# Autodesk Inventor assembly: s-assy-base_light
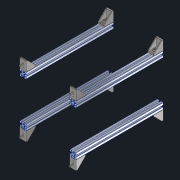
[picture p0: Inventor's stored thumbnail of the model, 180x180]
Saved by Autodesk Inventor 2022 (Build 260153000, 153)
## iProperties
Created: 2021-10-19
Part Number: s-assy-base_light
Document SubType Name: Assembly
Designer: Yuta Kage
Mass: 997.591 g
Surface Area: 2388.51 cm^2
Volume: 260.269 cm^3
Density: 3.83292 g/cm^3
Author: Yuta Kage
## Documents named in this file (4)
- C:\Users\yuta0\Documents\GitHub\catchrobo_hardware\assy-scara\s-assy-base_light.iam
- C:\Users\yuta0\Documents\GitHub\catchrobo_hardware\assy-scara\NFS5-2020_1.ipt
- C:\Users\yuta0\Documents\GitHub\catchrobo_hardware\assy-scara\s-assy-blacket2.iam
- C:\Users\yuta0\Documents\GitHub\catchrobo_hardware\assy-scara\CB5-15.ipt
## Components (16 placed, 3 different names)
1. CB5-15:1
2. CB5-15:2
3. CB5-15:3
4. CB5-15:4
5. s-assy-blacket2:2 [sub-assembly] — メイト:19, フラッシュ:25, フラッシュ:26
6. NFS5-2020_1:5 — メイト:18, フラッシュ:23, フラッシュ:24, メイト:19, フラッシュ:25, フラッシュ:26
7. s-assy-blacket2:1 [sub-assembly] — メイト:18, フラッシュ:23, フラッシュ:24
8. NFS5-2020_1:3 — フラッシュ:28, メイト:21, フラッシュ:29, フラッシュ:30, メイト:25, フラッシュ:31
9. s-assy-blacket2:3 [sub-assembly] — フラッシュ:28, メイト:25, フラッシュ:31
10. s-assy-blacket2:7 [sub-assembly] — メイト:21, フラッシュ:29, フラッシュ:30
11. s-assy-blacket2:8 [sub-assembly]
12. NFS5-2020_1:6
13. s-assy-blacket2:9 [sub-assembly]
14. NFS5-2020_1:7
15. s-assy-blacket2:10 [sub-assembly]
16. s-assy-blacket2:11 [sub-assembly]
## Component patterns: (4 elements, first: CB5-15:1), (2 elements, first: s-assy-blacket2:2 + NFS5-2020_1:5 + s-assy-blacket2:1 + NFS5-2020_1:3 + s-assy-blacket2:3 + s-assy-blacket2:7)
## Relationships (12: Flush 8, Mate 4)
- メイト:18 [Mate]: NFS5-2020_1:5 ↔ s-assy-blacket2:1
- フラッシュ:23 [Flush]: NFS5-2020_1:5 ↔ s-assy-blacket2:1
- フラッシュ:24 [Flush]: NFS5-2020_1:5 ↔ s-assy-blacket2:1
- メイト:19 [Mate]: s-assy-blacket2:2 ↔ NFS5-2020_1:5
- フラッシュ:25 [Flush]: s-assy-blacket2:2 ↔ NFS5-2020_1:5
- フラッシュ:26 [Flush]: s-assy-blacket2:2 ↔ NFS5-2020_1:5
- フラッシュ:28 [Flush]: NFS5-2020_1:3 ↔ s-assy-blacket2:3
- メイト:21 [Mate]: NFS5-2020_1:3 ↔ s-assy-blacket2:7
- フラッシュ:29 [Flush]: NFS5-2020_1:3 ↔ s-assy-blacket2:7
- フラッシュ:30 [Flush]: NFS5-2020_1:3 ↔ s-assy-blacket2:7
- メイト:25 [Mate]: NFS5-2020_1:3 ↔ s-assy-blacket2:3
- フラッシュ:31 [Flush]: NFS5-2020_1:3 ↔ s-assy-blacket2:3
